# Autodesk Inventor assembly: Motor Panel
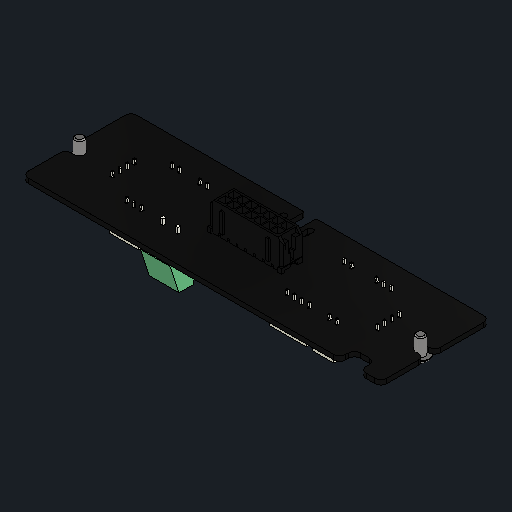
[picture p0: Inventor's stored thumbnail of the model, 512x512]
Saved by Autodesk Inventor 2025.1 (Build 291241020, 241B)
## iProperties
Created: 2025-05-09
Part Number: Motor Panel
Document SubType Name: Assembly
Designer: AdminForWorker
Title: Motor Panel
Author: AdminForWorker
## Documents named in this file (3)
- C:\Users\Joshua Eah\Documents\Voron 0.2\CAD\Master Assembly\Panels\Motor Panel.iam
- C:\Users\Joshua Eah\Documents\Voron 0.2\CAD\Master Assembly\Panels\Umbilical Panel\V0-UmbilicalBoardRevA.iam
- C:\Users\Joshua Eah\Documents\Voron 0.2\CAD\Master Assembly\Hardware\M3x6 BHCS.ipt
## Components (3 placed, 2 different names)
1. V0-UmbilicalBoardRevA:1 [sub-assembly] — Mate:1, Mate:2, Mate:3
2. M3x6 BHCS:7 — Mate:1, Mate:3
3. M3x6 BHCS:8 — Mate:2
## Relationships (3: Mate 3)
- Mate:1: V0-UmbilicalBoardRevA:1 ↔ M3x6 BHCS:7
- Mate:2: V0-UmbilicalBoardRevA:1 ↔ M3x6 BHCS:8
- Mate:3: V0-UmbilicalBoardRevA:1 ↔ M3x6 BHCS:7
